# Autodesk Inventor assembly: Hexapod
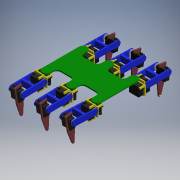
[picture p0: Inventor's stored thumbnail of the model, 180x180]
Saved by Autodesk Inventor 2017 (Build 210142000, 142)
## iProperties
Part Number: Hexapod
Document SubType Name: Assembly
Designer: Alexander Miller
Author: Alexander Miller
## Documents named in this file (3)
- D:\Alexander Miller\Documents\Git\Hexapod\3DParts\Hexapod.iam
- D:\Alexander Miller\Documents\Git\Hexapod\3DParts\Body_bottom.ipt
- D:\Alexander Miller\Documents\Git\Hexapod\3DParts\leg.iam
## Components (7 placed, 2 different names)
1. Body_bottom:1 — Rigid:1, Rigid:2, Rigid:3, Rigid:4, Rigid:5, Rigid:6
2. leg:1 [sub-assembly] — Rigid:1
3. leg:2 [sub-assembly] — Rigid:6
4. leg:3 [sub-assembly] — Rigid:2
5. leg:4 [sub-assembly] — Rigid:5
6. leg:5 [sub-assembly] — Rigid:3
7. leg:6 [sub-assembly] — Rigid:4
## Relationships (6: WeldJoint 6)
- Rigid:1 [WeldJoint]: Body_bottom:1 ↔ leg:1
- Rigid:2 [WeldJoint]: Body_bottom:1 ↔ leg:3
- Rigid:3 [WeldJoint]: Body_bottom:1 ↔ leg:5
- Rigid:4 [WeldJoint]: Body_bottom:1 ↔ leg:6
- Rigid:5 [WeldJoint]: Body_bottom:1 ↔ leg:4
- Rigid:6 [WeldJoint]: Body_bottom:1 ↔ leg:2
